# Autodesk Inventor assembly: servoMount
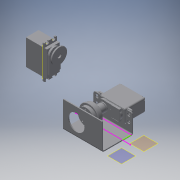
[picture p0: Inventor's stored thumbnail of the model, 180x180]
Saved by Autodesk Inventor 2017 (Build 210142000, 142)
## iProperties
Created: 2017-03-22
Part Number: servoMount
Document SubType Name: Assembly
Designer: admin
Author: admin
## Documents named in this file (6)
- C:\Users\admin\Desktop\CAD\servoMount.iam
- C:\Users\admin\Downloads\bearing.ipt
- C:\Users\admin\Downloads\hub.ipt
- C:\Users\admin\Desktop\CAD\HS-322HD.ipt
- C:\Users\admin\Downloads\Hitec HS-325HB.ipt
- C:\Users\admin\Desktop\CAD\HSmount.ipt
## Components (5 placed, 5 different names)
1. bearing:1 — Rigid:1
2. hub:1 — Rigid:1, Insert:1
3. HS-322HD:1
4. Hitec HS-325HB:1 — Insert:1, Mate:1, Mate:2
5. HSmount:1 — Mate:1, Mate:2
## Relationships (4: Mate 2, WeldJoint 1, Insert 1)
- Rigid:1 [WeldJoint]: bearing:1 ↔ hub:1
- Insert:1: hub:1 ↔ Hitec HS-325HB:1
- Mate:1: Hitec HS-325HB:1 ↔ HSmount:1
- Mate:2: Hitec HS-325HB:1 ↔ HSmount:1
